# Autodesk Inventor assembly: MotorBlockOneWheel
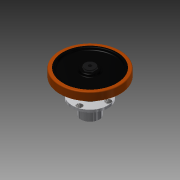
[picture p0: Inventor's stored thumbnail of the model, 180x180]
Saved by Autodesk Inventor 2014 SP1 (Build 180222100, 222)
## iProperties
Created: 2015-04-11
Part Number: MotorBlockOneWheel
Document SubType Name: Assembly
Designer: david
Mass: 101.366 g
Surface Area: 228.874 cm^2
Volume: 43.1349 cm^3
Density: 2.34997 g/cm^3
Author: david
## Documents named in this file (3)
- C:\Users\asus\Documents\Autodesk\Projects\AUSBEEDone\Components\Motors\MotorBlockOneWheel.iam
- C:\Users\asus\Documents\Autodesk\Projects\AUSBEEDone\Components\Motors\Motor.iam
- C:\Users\asus\Documents\Autodesk\Projects\AUSBEEDone\Components\BaneBots\OneWheelBlock.iam
## Components (2 placed, 2 different names)
1. Motor:1 [sub-assembly] — Mate:1, Insert:1, Mate:2, Angle:1
2. OneWheelBlock:1 [sub-assembly] — Mate:1, Insert:1, Mate:2, Angle:1
## Relationships (4: Mate 2, Insert 1, Angle 1)
- Mate:1: Motor:1 ↔ OneWheelBlock:1
- Insert:1: Motor:1 ↔ OneWheelBlock:1
- Mate:2: Motor:1 ↔ OneWheelBlock:1
- Angle:1 (0 deg): Motor:1 ↔ OneWheelBlock:1
